# Autodesk Inventor assembly: RIGHTRIGHTzmotorblock
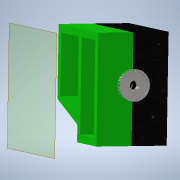
[picture p0: Inventor's stored thumbnail of the model, 180x180]
Saved by Autodesk Inventor 2020 (Build 240168000, 168)
## iProperties
Created: 2021-02-28
Part Number: RIGHTRIGHTzmotorblock
Document SubType Name: Assembly
Designer: AOB
Mass: 120.624 g
Surface Area: 407.974 cm^2
Volume: 82.7913 cm^3
Density: 1.45697 g/cm^3
Author: AOB
## Documents named in this file (5)
- C:\Users\marti\Documents\Inventor\ProjectBoron\ultimate boron\RIGHTRIGHTzmotorblock.iam
- RIGHTzmotorblock.iam
- C:\Users\marti\Documents\Inventor\ProjectBoron\ultimate boron\RIGHTzmotorblockleft-half.ipt
- C:\Users\marti\Documents\Inventor\ProjectBoron\ultimate boron\RIGHTzmotorblockright-half.ipt
- C:\Users\marti\Documents\Inventor\ProjectBoron\ultimate boron\RIGHTflange-bearing.ipt
## Components (5 placed, 3 different names)
1. RIGHTzmotorblockleft-half:1 — Flush:3, Flush:2, Flush:1, Rigid:1
2. RIGHTzmotorblockright-half:1 — Flush:3, Flush:2, Flush:1, Mate:3, Mate:2, Mate:5, Mate:4, Mate:7, Mate:6, Flush:4, Rigid:1
3. RIGHTflange-bearing:1 — Mate:3, Mate:2
4. RIGHTflange-bearing:2 — Mate:5, Mate:4
5. RIGHTflange-bearing:3 — Mate:7, Mate:6
## Relationships (11: Mate 6, Flush 4, WeldJoint 1)
- Flush:3: RIGHTzmotorblockleft-half:1 ↔ RIGHTzmotorblockright-half:1
- Flush:2: RIGHTzmotorblockleft-half:1 ↔ RIGHTzmotorblockright-half:1
- Flush:1: RIGHTzmotorblockleft-half:1 ↔ RIGHTzmotorblockright-half:1
- Mate:3: RIGHTzmotorblockright-half:1 ↔ RIGHTflange-bearing:1
- Mate:2: RIGHTzmotorblockright-half:1 ↔ RIGHTflange-bearing:1
- Mate:5: RIGHTzmotorblockright-half:1 ↔ RIGHTflange-bearing:2
- Mate:4: RIGHTzmotorblockright-half:1 ↔ RIGHTflange-bearing:2
- Mate:7: RIGHTzmotorblockright-half:1 ↔ RIGHTflange-bearing:3
- Mate:6: RIGHTzmotorblockright-half:1 ↔ RIGHTflange-bearing:3
- Flush:4 (30 mm): RIGHTzmotorblockright-half:1
- Rigid:1 [WeldJoint]: RIGHTzmotorblockleft-half:1 ↔ RIGHTzmotorblockright-half:1
